# Autodesk Inventor assembly: ElvEndEffectFrame
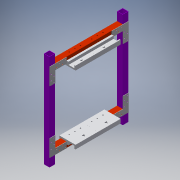
[picture p0: Inventor's stored thumbnail of the model, 180x180]
Saved by Autodesk Inventor 2019 (Build 230136000, 136)
## iProperties
Created: 2019-01-10
Part Number: ElvEndEffectFrame
Document SubType Name: Assembly
Designer: james
Mass: 912.548 g
Surface Area: 3456.75 cm^2
Volume: 461.794 cm^3
Density: 1.97609 g/cm^3
Author: james
## Documents named in this file (5)
- F:\JimsDesign\2019CHS4089\ElvEndEffectFrame.iam
- F:\JimsDesign\2019CHS4089\ElvCrossBeam.ipt
- F:\JimsDesign\2019CHS4089\ElvEndEffectBeam.ipt
- F:\JimsDesign\2019CHS4089\elvRivetPlate.ipt
- F:\JimsDesign\2019CHS4089\ElvDelV5.ipt
## Components (12 placed, 4 different names)
1. ElvCrossBeam:1 — Mate:31, Mate:32, Mate:33, Mate:34, Mate:41, Mate:43, Mate:44, Mate:45, Mate:46, Mate:47, Mate:57, Mate:58
2. ElvCrossBeam:2 — Mate:7, Mate:8, Mate:10, Mate:11, Mate:42, Mate:48, Mate:49, Mate:50, Mate:51, Mate:52, Mate:53, Mate:59, Mate:60
3. ElvEndEffectBeam:1 — Mate:35, Mate:36, Mate:37, Mate:38, Mate:39, Mate:40
4. ElvEndEffectBeam:2 — Mate:54, Mate:55, Mate:56
5. ElvDelV5:1 — Mate:31, Mate:32, Mate:57
6. ElvDelV5:2 — Mate:7, Mate:8, Mate:59
7. ElvDelV5:3 — Mate:33, Mate:34, Mate:58
8. ElvDelV5:4 — Mate:10, Mate:11, Mate:60
9. elvRivetPlate:1 — Mate:45, Mate:46, Mate:47, Mate:56
10. elvRivetPlate:2 — Mate:38, Mate:39, Mate:40, Mate:42, Mate:51, Mate:52, Mate:53
11. elvRivetPlate:3 — Mate:35, Mate:36, Mate:37, Mate:41, Mate:43, Mate:44
12. elvRivetPlate:4 — Mate:48, Mate:49, Mate:50, Mate:54, Mate:55
## Relationships (34: Mate 34)
- Mate:7: ElvCrossBeam:2 ↔ ElvDelV5:2
- Mate:8: ElvCrossBeam:2 ↔ ElvDelV5:2
- Mate:10: ElvCrossBeam:2 ↔ ElvDelV5:4
- Mate:11: ElvCrossBeam:2 ↔ ElvDelV5:4
- Mate:31: ElvCrossBeam:1 ↔ ElvDelV5:1
- Mate:32: ElvCrossBeam:1 ↔ ElvDelV5:1
- Mate:33: ElvCrossBeam:1 ↔ ElvDelV5:3
- Mate:34: ElvCrossBeam:1 ↔ ElvDelV5:3
- Mate:35: ElvEndEffectBeam:1 ↔ elvRivetPlate:3
- Mate:36: ElvEndEffectBeam:1 ↔ elvRivetPlate:3
- Mate:37: ElvEndEffectBeam:1 ↔ elvRivetPlate:3
- Mate:38: ElvEndEffectBeam:1 ↔ elvRivetPlate:2
- Mate:39: ElvEndEffectBeam:1 ↔ elvRivetPlate:2
- Mate:40: ElvEndEffectBeam:1 ↔ elvRivetPlate:2
- Mate:41: ElvCrossBeam:1 ↔ elvRivetPlate:3
- Mate:42: ElvCrossBeam:2 ↔ elvRivetPlate:2
- Mate:43: ElvCrossBeam:1 ↔ elvRivetPlate:3
- Mate:44: ElvCrossBeam:1 ↔ elvRivetPlate:3
- Mate:45: ElvCrossBeam:1 ↔ elvRivetPlate:1
- Mate:46: ElvCrossBeam:1 ↔ elvRivetPlate:1
- Mate:47: ElvCrossBeam:1 ↔ elvRivetPlate:1
- Mate:48: ElvCrossBeam:2 ↔ elvRivetPlate:4
- Mate:49: ElvCrossBeam:2 ↔ elvRivetPlate:4
- Mate:50: ElvCrossBeam:2 ↔ elvRivetPlate:4
- Mate:51: ElvCrossBeam:2 ↔ elvRivetPlate:2
- Mate:52: ElvCrossBeam:2 ↔ elvRivetPlate:2
- Mate:53: ElvCrossBeam:2 ↔ elvRivetPlate:2
- Mate:54: ElvEndEffectBeam:2 ↔ elvRivetPlate:4
- Mate:55: ElvEndEffectBeam:2 ↔ elvRivetPlate:4
- Mate:56: ElvEndEffectBeam:2 ↔ elvRivetPlate:1
- Mate:57: ElvCrossBeam:1 ↔ ElvDelV5:1
- Mate:58: ElvCrossBeam:1 ↔ ElvDelV5:3
- Mate:59: ElvCrossBeam:2 ↔ ElvDelV5:2
- Mate:60: ElvCrossBeam:2 ↔ ElvDelV5:4
